# Autodesk Inventor assembly: FootRightNCS
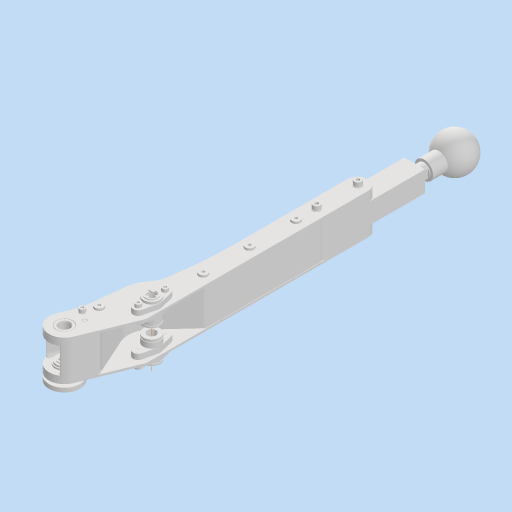
[picture p0: Inventor's stored thumbnail of the model, 512x512]
Saved by Autodesk Inventor 2023 (Build 270158000, 158)
## iProperties
Created: 2026-06-19
Part Number: FootRightNCS
Document SubType Name: Assembly
Designer: Nathann
Author: Nathann
## Documents named in this file (2)
- C:\Users\Nathann\ClawdDrive\Objet3D\RunningRobot\PartURDF\FootRightNCS.iam
- C:\Users\Nathann\ClawdDrive\Objet3D\RunningRobot\PartURDF\FootRight.iam
## Components (1 placed, 1 different names)
1. FootRight:1 [sub-assembly] — Mate:1, Flush:1, Flush:2, Angle:1
## Relationships (8: Mate 4, Flush 2, Symmetry 1, Angle 1)
- Mate:1: FootRight:1
- Mate:2
- Mate:3
- Flush:1: FootRight:1
- Flush:2: FootRight:1
- Symmetry:1
- Mate:4
- Angle:1 (0 deg): FootRight:1
